# Autodesk Inventor assembly: Assembly1
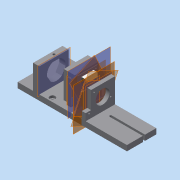
[picture p0: Inventor's stored thumbnail of the model, 180x180]
Saved by Autodesk Inventor 2019.4 (Build 234330000, 330)
## iProperties
Created: 2020-12-23
Part Number: Assembly1
Document SubType Name: Assembly
Designer: diederichbenedict
Author: diederichbenedict
## Documents named in this file (4)
- C:\Users\diederichbenedict\Dropbox\Dokumente\Promotion\PROJECTS\STORMoChip\GITHUB\CAD\cellSTORM_inverted\Workspace\Assembly1.iam
- C:\Users\diederichbenedict\Dropbox\Dokumente\Promotion\PROJECTS\STORMoChip\GITHUB\CAD\cellSTORM_inverted\Workspace\cellSTORM_inverted_Laser_10x_laserscanner_left_v2.ipt
- C:\Users\diederichbenedict\Dropbox\Dokumente\Promotion\PROJECTS\STORMoChip\GITHUB\CAD\cellSTORM_inverted\Workspace\00_KES400.iam
- C:\Users\diederichbenedict\Dropbox\Dokumente\Promotion\PROJECTS\STORMoChip\GITHUB\CAD\cellSTORM_inverted\Workspace\cellSTORM_inverted_spacerblock_KES400.ipt
## Components (4 placed, 3 different names)
1. cellSTORM_inverted_Laser_10x_laserscanner_left_v2:1 — Insert:1, Angle:1, Angle:2, Flush:1, Flush:2
2. 00_KES400:1 [sub-assembly] — Insert:1, Angle:1, Insert:2
3. 00_KES400:2 [sub-assembly] — Insert:2, Angle:2
4. cellSTORM_inverted_spacerblock_KES400:1 — Flush:1, Flush:2
## Relationships (6: Insert 2, Angle 2, Flush 2)
- Insert:1: cellSTORM_inverted_Laser_10x_laserscanner_left_v2:1 ↔ 00_KES400:1
- Angle:1 (0 deg): cellSTORM_inverted_Laser_10x_laserscanner_left_v2:1 ↔ 00_KES400:1
- Insert:2 (2 mm): 00_KES400:1 ↔ 00_KES400:2
- Angle:2 (0 deg): cellSTORM_inverted_Laser_10x_laserscanner_left_v2:1 ↔ 00_KES400:2
- Flush:1: cellSTORM_inverted_Laser_10x_laserscanner_left_v2:1 ↔ cellSTORM_inverted_spacerblock_KES400:1
- Flush:2: cellSTORM_inverted_Laser_10x_laserscanner_left_v2:1 ↔ cellSTORM_inverted_spacerblock_KES400:1
